# Autodesk Inventor assembly: FullCaseWithBaccable
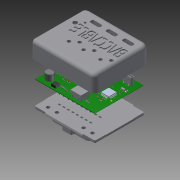
[picture p0: Inventor's stored thumbnail of the model, 180x180]
Saved by Autodesk Inventor 2014 SP2 (Build 180246200, 246)
## iProperties
Created: 2025-02-22
Part Number: FullCaseWithBaccable
Document SubType Name: Assembly
Designer: GauchoHP
Author: GauchoHP
## Documents named in this file (6)
- G:\Dati\Documenti_Emanuele\Linguaggi_di_Programmazione\ST MCU\baccable\canable\BACCAble-master\hardware\box\baccable_lastest_case_for_new_PCB_V2\FullCaseWithBaccable.iam
- FullCaseWithBaccableV2.iam
- G:\Dati\Documenti_Emanuele\Linguaggi_di_Programmazione\ST MCU\baccable\canable\BACCAble-master\hardware\box\baccable_lastest_case_for_new_PCB_V2\obdBase.ipt
- G:\Dati\Documenti_Emanuele\Linguaggi_di_Programmazione\ST MCU\baccable\canable\BACCAble-master\hardware\box\baccable_lastest_case_for_new_PCB_V2\cover.ipt
- G:\Dati\Documenti_Emanuele\Linguaggi_di_Programmazione\ST MCU\baccable\canable\nuovo progetto PCB\baccable\Imported Components\BaccableNew\BaccableNew.iam
- G:\Dati\Documenti_Emanuele\Linguaggi_di_Programmazione\ST MCU\baccable\canable\BACCAble-master\hardware\box\baccable_lastest_case_for_new_PCB_V2\Imported Components\0510210200\0510210200.ipt
## Components (4 placed, 4 different names)
1. cover:1 — Mate:8, Mate:9
2. BaccableNew:1 [sub-assembly] — Mate:6, Mate:7, Mate:10, Mate:11
3. obdBase:2 — Mate:6, Mate:7, Mate:8, Mate:9
4. 0510210200:1 — Mate:10, Mate:11
## Relationships (6: Mate 6)
- Mate:6 (0.2 mm): BaccableNew:1 ↔ obdBase:2
- Mate:7 (0.2 mm): BaccableNew:1 ↔ obdBase:2
- Mate:8 (0.3 mm): cover:1 ↔ obdBase:2
- Mate:9 (0.3 mm): cover:1 ↔ obdBase:2
- Mate:10: BaccableNew:1 ↔ 0510210200:1
- Mate:11: BaccableNew:1 ↔ 0510210200:1
